# Autodesk Inventor assembly: Baumer_OXS200_11728845_1
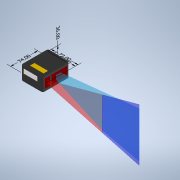
[picture p0: Inventor's stored thumbnail of the model, 180x180]
Saved by Autodesk Inventor 2021 (Build 250183000, 183)
## iProperties
Category: PARTsolutions
Company: BAUMER
Created: 2025-06-20
Part Number: Baumer_OXS200_11728845_1
Catalog Web Link: www.cadenas.de
Description: OX-Smart profile sensors
Vendor: BAUMER
Document SubType Name: Assembly
Designer: psAdmin
Manufacturer: BAUMER
Mass: 270 g
Surface Area: 1027.7 cm^2
Volume: 345.906 cm^3
Density: 0.78056 g/cm^3
Title: OXS200-R10A.E02
Author: Cadenas PARTsolutions
Comments: Smart profile sensors
PSOL_IDENT_0: {$CADENAS_DATA/23d-libs/baumer/products/smartvisionsensors/smartprofilesensors/oxmp/oxmp_asmtab.prj}
PSOL_IDENT_1: ,194 {VTYP=3D},{STYP=ASSTAB},{NB=Baumer_OXS200_11728845_1},{LINA=OXS200-R10A.E02},{NN=OX},{DATE=12.0
PSOL_IDENT_2: 6.2025 11:29:18},{GEOMDATE=06.05.2025 06:41:05},{VERSION=},{LINEID=250},{WBVAR=AG},{WBNUMERIC=AG}  {
PSOL_IDENT_3: NB=Baumer_OXS200_11728845_1},{LINA=OXS200-R10A.E02},{KT=DUMMY},{TYPE=Measuring mode (E): Edge, Width
PSOL_IDENT_4: /Gap, Intensity Edge, Segment Selector, Caliper X/Z/Distance},{LWL=Red (660 nm)},{MR=100},{TC=OXS200
PSOL_IDENT_5: -R10A.E02},{TCX=OXS200},{AN=11728845},{AG=1},{WS=icon_website.png},{PD=https://www.baumer.com/pid/11
PSOL_IDENT_6: 728845},{EP=eplan_data_standard.png},{EPL=https://dataportal.eplan.com/part-details/bau.11728845},{M
PSOL_IDENT_7: H=Aluminium},{MO=Glass},{WT=270},{PC=IP 65},{LC=2},{ET=18 … 30 VDC},{AOS=4-20mA, 2-10mA, 0-10V, 0-5V
PSOL_IDENT_8: },{SO=2 x Outputs (Push-Pull)},{CONS=typ. 2.4W (100 mA max at 24 V) | IEEE 802.3af Power over Ethern
PSOL_IDENT_9: et (PoE)},{OT=0 ... + 45 °C},{ALI=< 25 kLux},{CS=CE, UL, PROFINET, ETHERNET/IP},{EC=t.b.d.},{CTN=t.b
PSOL_IDENT_10: .d.},{COO=t.b.d.},{TYPEX=1},{LWLX=1},{B0=7.500},{H0=3.000},{SDC=150.000},{B1=75.000},{H1=0.650},{B2=
PSOL_IDENT_11: 125.000},{H2=0.750},{EH=8.500},{RH=37.300},{RW=12.000},{HX=0.400},{L2=250.000},{PPATH=oxmp_asmtpl.pr
PSOL_IDENT_12: j},{VIS=1}
NB: Baumer_OXS200_11728845_1
NN: OX
NT: Smart profile sensors
NBSYN: Baumer_$TCX._$AN._$AG.
LINA: OXS200-R10A.E02
CATALOG: Baumer Group
TYPE: Measuring mode (E): Edge, Width/Gap, Intensity Edge, Segment Selector, Caliper X/Z/Distance
LWL: Red (660 nm)
MR: 100
TC: OXS200-R10A.E02
AN: 11728845
AG: nominal beam
WS: icon_website.png
EP: eplan_data_standard.png
MH: aluminium
MO: Glass
WT: 270
PC: IP 65
LC: 2
ET: 18 ... 30 VDC
AOS: 4 ... 20 mA / 2 ... 10 mA / 0 ... 10 VDC / 0 ... 5 VDC
SO: 2 x Outputs (Push-Pull)
CONS: typ. 2.4W (100 mA max at 24 V) | IEEE 802.3af Power over Ethernet (PoE)
OT: 0 ... +45 °C
ALI: < 25 kLux
CS: CE, UL, PROFINET, ETHERNET/IP
SUPPLIER: BAUMER
ARTICLENO: Baumer_OXS200_11728845_1
BOMINFO: OXS200-R10A.E02
CREATOR: CADENAS GmbH
## Documents named in this file (5)
- e:\temp\worker_COMMON_242\temp\tmp_7844_78_51UKp\format_0\Baumer_OXS200_11728845_1.iam
- e:\temp\worker_COMMON_242\temp\tmp_7844_78_51UKp\format_0\3D_OXS200_11728845.ipt
- e:\temp\worker_COMMON_242\temp\tmp_7844_78_51UKp\format_0\Blindrange_OXS200_11728845.ipt
- e:\temp\worker_COMMON_242\temp\tmp_7844_78_51UKp\format_0\Measuringrange_OXS200_11728845.ipt
- e:\temp\worker_COMMON_242\temp\tmp_7844_78_51UKp\format_0\Receivingbeam_OXS200_11728845.ipt
## Components (4 placed, 4 different names)
1. 3D_OXS200_11728845:1 — CP2_XY@1 <-> CP1_XY@2, CP2_Z@1 <-> CP1_Z@2, CP2_YZ@1 <-> CP1_YZ@2, CP2_XY@1 <-> CP1_XY@3, CP2_Z@1 <-> CP1_Z@3, CP2_YZ@1 <-> CP1_YZ@3, CP2_XY@1 <-> CP1_XY@4, CP2_Z@1 <-> CP1_Z@4, CP2_YZ@1 <-> CP1_YZ@4
2. Blindrange_OXS200_11728845:1 — CP2_XY@1 <-> CP1_XY@2, CP2_Z@1 <-> CP1_Z@2, CP2_YZ@1 <-> CP1_YZ@2
3. Measuringrange_OXS200_11728845:1 — CP2_XY@1 <-> CP1_XY@3, CP2_Z@1 <-> CP1_Z@3, CP2_YZ@1 <-> CP1_YZ@3
4. Receivingbeam_OXS200_11728845:1 — CP2_XY@1 <-> CP1_XY@4, CP2_Z@1 <-> CP1_Z@4, CP2_YZ@1 <-> CP1_YZ@4
## Relationships (9: Flush 3, Mate 3, Angle 3)
- CP2_XY@1 <-> CP1_XY@2 [Flush]: 3D_OXS200_11728845:1 ↔ Blindrange_OXS200_11728845:1
- CP2_Z@1 <-> CP1_Z@2 [Mate]: 3D_OXS200_11728845:1 ↔ Blindrange_OXS200_11728845:1
- CP2_YZ@1 <-> CP1_YZ@2 [Angle] (0 deg): 3D_OXS200_11728845:1 ↔ Blindrange_OXS200_11728845:1
- CP2_XY@1 <-> CP1_XY@3 [Flush]: 3D_OXS200_11728845:1 ↔ Measuringrange_OXS200_11728845:1
- CP2_Z@1 <-> CP1_Z@3 [Mate]: 3D_OXS200_11728845:1 ↔ Measuringrange_OXS200_11728845:1
- CP2_YZ@1 <-> CP1_YZ@3 [Angle] (0 deg): 3D_OXS200_11728845:1 ↔ Measuringrange_OXS200_11728845:1
- CP2_XY@1 <-> CP1_XY@4 [Flush]: 3D_OXS200_11728845:1 ↔ Receivingbeam_OXS200_11728845:1
- CP2_Z@1 <-> CP1_Z@4 [Mate]: 3D_OXS200_11728845:1 ↔ Receivingbeam_OXS200_11728845:1
- CP2_YZ@1 <-> CP1_YZ@4 [Angle] (0 deg): 3D_OXS200_11728845:1 ↔ Receivingbeam_OXS200_11728845:1
